# Autodesk Inventor assembly: ASM_Micron_Rev2_ASAP_FPCB
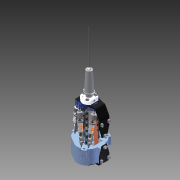
[picture p0: Inventor's stored thumbnail of the model, 180x180]
Saved by Autodesk Inventor 2011 SP2 (Build 150309200, 309)
## iProperties
Created: 2012-01-18
Part Number: ASM_Micron_Rev2_ASAP_FPCB
Document SubType Name: Assembly
Designer: sungwook
Author: sungwook
## Documents named in this file (12)
- C:\Users\sungwook\Documents\Inventor\Micron22_top_adj_02082013\Assembly\ASM_Micron_Rev2_ASAP_FPCB.iam
- C:\Users\sungwook\Documents\Inventor\Micron22_top_adj_02082013\Parts\Main\Platform_Base_20mm_Rev2.ipt
- C:\Users\sungwook\Documents\Inventor\Micron22_top_adj_02082013\Parts\Main\Platform_Top_14mm_Rev.ipt
- C:\Users\sungwook\Documents\Inventor\Micron22_top_adj_02082013\Parts\Tool\ASM_Tool_Tip_Rev.iam
- C:\Users\sungwook\Documents\Inventor\Micron22_top_adj_02082013\Assembly\ASM_Motor_Unit_Rev.iam
- C:\Users\sungwook\Documents\Inventor\Micron22_top_adj_02082013\Parts\Main\Eye_Pin_26Ga.ipt
- C:\Users\sungwook\Documents\Inventor\Content Center Files\R2011\en-US\ANSI B18.6.3(12)\ANSI B18.6.3 - 0-80 UNF - 0.1875(15_).ipt
- C:\Users\sungwook\Documents\Inventor\Micron22_top_adj_02082013\Parts\Main\Spring.ipt
- C:\Users\sungwook\Documents\Inventor\Micron22_top_adj_02082013\Parts\ASAP\Handle_ASAP.iam
- C:\Users\sungwook\Documents\Inventor\Micron22_top_adj_02082013\Parts\ASAP\Platform_ASAP.iam
- C:\Users\sungwook\Documents\Inventor\Micron22_top_adj_02082013\Parts\Main\Guide Tube.ipt
- C:\Users\sungwook\Documents\Inventor\Micron22_top_adj_02082013\Parts\Main\FPCB_1.ipt
## Components (25 placed, 11 different names)
1. Platform_Base_20mm_Rev2:1 — Mate:4, Mate:6, Mate:8, Angle:1, Mate:29, Mate:30, Mate:31, Mate:32, Flush:23, Mate:33, Mate:35, Mate:38
2. Platform_Top_14mm_Rev:1 — Mate:1, Mate:2, Mate:3, Mate:4, Mate:5, Mate:7, Angle:1, Mate:9, Mate:10, Angle:2, Mate:18, Mate:22
3. ASM_Tool_Tip_Rev:1 [sub-assembly] — Mate:1, Mate:2, Mate:3, Mate:11, Mate:20
4. Handle_ASAP:1 [sub-assembly] — Flush:1, Mate:29, Mate:30, Mate:31, Mate:38
5. Platform_ASAP:1 [sub-assembly] — Mate:16, Mate:17, Mate:18, Mate:21
6. Guide Tube:1 — Mate:20, Mate:21
7. FPCB_1:1 — Flush:22, Mate:22
8. ASM_Motor_Unit_Rev:1 [sub-assembly] — Mate:5, Mate:6
9. ASM_Motor_Unit_Rev:2 [sub-assembly] — Mate:7, Mate:8
10. ASM_Motor_Unit_Rev:3 [sub-assembly]
11. ASM_Motor_Unit_Rev:4 [sub-assembly]
12. ASM_Motor_Unit_Rev:5 [sub-assembly]
13. ASM_Motor_Unit_Rev:6 [sub-assembly]
14. Cross Recessed Flat Countersunk Head Machine Screw - Type I - Inch 0-80 x 3/16:1 — Mate:11, Mate:16
15. Cross Recessed Flat Countersunk Head Machine Screw - Type I - Inch 0-80 x 3/16:2
16. Cross Recessed Flat Countersunk Head Machine Screw - Type I - Inch 0-80 x 3/16:3 — Mate:17
17. Eye_Pin_26Ga:1 — Mate:9, Mate:10, Angle:2, Mate:34, Mate:36, Mate:37
18. Spring:1 — Mate:33, Mate:34, Mate:35, Mate:36, Mate:37
19. Eye_Pin_26Ga:4 — Mate:32, Flush:23
20. Eye_Pin_26Ga:5
21. Spring:2
22. Eye_Pin_26Ga:6
23. Eye_Pin_26Ga:7
24. Spring:3
25. Eye_Pin_26Ga:8
## Component patterns: (3 elements, first: ASM_Motor_Unit_Rev:1 + ASM_Motor_Unit_Rev:2), Tool Mount Bolts (3 elements), Spring (3 elements)
## Relationships (32: Mate 27, Flush 3, Angle 2)
- Mate:1: Platform_Top_14mm_Rev:1 ↔ ASM_Tool_Tip_Rev:1
- Mate:2: Platform_Top_14mm_Rev:1 ↔ ASM_Tool_Tip_Rev:1
- Mate:3: Platform_Top_14mm_Rev:1 ↔ ASM_Tool_Tip_Rev:1
- Mate:4: Platform_Base_20mm_Rev2:1 ↔ Platform_Top_14mm_Rev:1
- Mate:5: Platform_Top_14mm_Rev:1 ↔ ASM_Motor_Unit_Rev:1
- Mate:6: Platform_Base_20mm_Rev2:1 ↔ ASM_Motor_Unit_Rev:1
- Mate:7: Platform_Top_14mm_Rev:1 ↔ ASM_Motor_Unit_Rev:2
- Mate:8: Platform_Base_20mm_Rev2:1 ↔ ASM_Motor_Unit_Rev:2
- Angle:1 (180 deg): Platform_Base_20mm_Rev2:1 ↔ Platform_Top_14mm_Rev:1
- Mate:9: Platform_Top_14mm_Rev:1 ↔ Eye_Pin_26Ga:1
- Mate:10: Platform_Top_14mm_Rev:1 ↔ Eye_Pin_26Ga:1
- Angle:2 (0 deg): Platform_Top_14mm_Rev:1 ↔ Eye_Pin_26Ga:1
- Mate:16: Platform_ASAP:1 ↔ Cross Recessed Flat Countersunk Head Machine Screw - Type I - Inch 0-80 x 3/16:1
- Mate:17: Platform_ASAP:1 ↔ Cross Recessed Flat Countersunk Head Machine Screw - Type I - Inch 0-80 x 3/16:3
- Mate:18: Platform_Top_14mm_Rev:1 ↔ Platform_ASAP:1
- Flush:1: Handle_ASAP:1
- Mate:20: ASM_Tool_Tip_Rev:1 ↔ Guide Tube:1
- Mate:21: Platform_ASAP:1 ↔ Guide Tube:1
- Flush:22: FPCB_1:1
- Mate:22: Platform_Top_14mm_Rev:1 ↔ FPCB_1:1
- Mate:29 (4.302 mm): Platform_Base_20mm_Rev2:1 ↔ Handle_ASAP:1
- Mate:30: Platform_Base_20mm_Rev2:1 ↔ Handle_ASAP:1
- Mate:31: Platform_Base_20mm_Rev2:1 ↔ Handle_ASAP:1
- Mate:32: Platform_Base_20mm_Rev2:1 ↔ Eye_Pin_26Ga:4
- Flush:23: Platform_Base_20mm_Rev2:1 ↔ Eye_Pin_26Ga:4
- Mate:33: Platform_Base_20mm_Rev2:1 ↔ Spring:1
- Mate:34: Eye_Pin_26Ga:1 ↔ Spring:1
- Mate:35: Platform_Base_20mm_Rev2:1 ↔ Spring:1
- Mate:36: Eye_Pin_26Ga:1 ↔ Spring:1
- Mate:37: Eye_Pin_26Ga:1 ↔ Spring:1
- Mate:38: Platform_Base_20mm_Rev2:1 ↔ Handle_ASAP:1
- Mate:11: ASM_Tool_Tip_Rev:1 ↔ Cross Recessed Flat Countersunk Head Machine Screw - Type I - Inch 0-80 x 3/16:1
